# Autodesk Inventor assembly: assembly.rev5
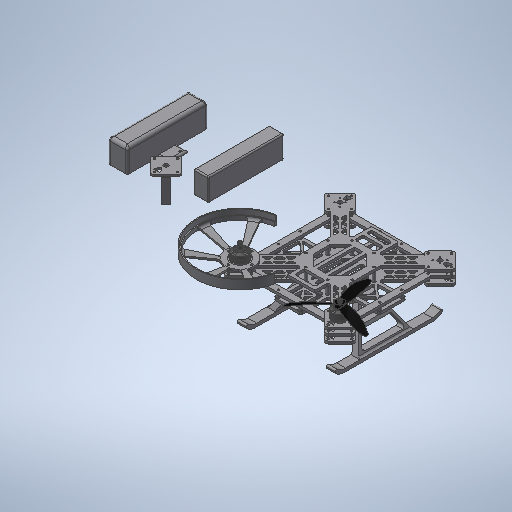
[picture p0: Inventor's stored thumbnail of the model, 512x512]
Saved by Autodesk Inventor 2025.2 (Build 292293000, 293)
## iProperties
Created: 2016-03-08
Part Number: assembly.rev5
Document SubType Name: Assembly
Designer: 200288284
Author: 200288284
## Documents named in this file (11)
- D:\UAV\机架\自制无人机\完整体.iam
- D:\UAV\机架\自制无人机\MOTOR_1806.iam
- D:\UAV\机架\自制无人机\Tri-Blade 5045 Propeller\Tri-Blade 5045 Propeller\5045 CCW.ipt
- D:\UAV\机架\自制无人机\电池.ipt
- D:\UAV\机架\自制无人机\Tri-Blade 5045 Propeller\Protection_for_2.5_inch_prop.ipt
- D:\UAV\机架\自制无人机\底板.ipt
- D:\UAV\机架\自制无人机\中版.ipt
- D:\UAV\机架\自制无人机\顶板.ipt
- D:\UAV\机架\自制无人机\起落架一体.ipt
- D:\UAV\机架\自制无人机\电池仓.ipt
- D:\UAV\机架\自制无人机\新起落架.ipt
## Components (13 placed, 10 different names)
1. 底板:1 — 配合:160, 配合:163, 配合:194, 配合:195, 表面齐平:1, 配合:196, 配合:197, 配合:199, 配合:200, 配合:201
2. 中版:1 — 配合:160, 配合:162, 配合:194, 配合:195
3. 顶板:1 — 配合:162, 配合:163, 配合:178, 配合:179, 配合:180, 配合:181, 配合:182, 配合:184, 配合:185, 配合:187, 配合:192, 配合:193
4. 电池:2 — 配合:192
5. MOTOR_1806:5 [sub-assembly] — 配合:180, 配合:181, 配合:183
6. Protection_for_2.5_inch_prop:5 — 配合:182, 配合:183, 配合:184
7. MOTOR_1806:8 [sub-assembly] — 配合:178, 配合:179, 配合:186, 配合:188, 配合:189
8. Protection_for_2.5_inch_prop:6 — 配合:185, 配合:186, 配合:187
9. 5045 CCW:5 — 配合:188, 配合:189
10. 电池仓:1 — 配合:193
11. 起落架一体:2
12. 新起落架:1 — 表面齐平:1, 配合:196, 配合:197
13. 新起落架:2 — 配合:199, 配合:200, 配合:201
## Relationships (25: Mate 24, Flush 1)
- 配合:160 [Mate]: 底板:1 ↔ 中版:1
- 配合:162 [Mate]: 中版:1 ↔ 顶板:1
- 配合:163 [Mate]: 底板:1 ↔ 顶板:1
- 配合:178 [Mate]: 顶板:1 ↔ MOTOR_1806:8
- 配合:179 [Mate]: 顶板:1 ↔ MOTOR_1806:8
- 配合:180 [Mate]: 顶板:1 ↔ MOTOR_1806:5
- 配合:181 [Mate]: 顶板:1 ↔ MOTOR_1806:5
- 配合:182 [Mate]: 顶板:1 ↔ Protection_for_2.5_inch_prop:5
- 配合:183 [Mate]: MOTOR_1806:5 ↔ Protection_for_2.5_inch_prop:5
- 配合:184 [Mate]: 顶板:1 ↔ Protection_for_2.5_inch_prop:5
- 配合:185 [Mate]: 顶板:1 ↔ Protection_for_2.5_inch_prop:6
- 配合:186 [Mate]: MOTOR_1806:8 ↔ Protection_for_2.5_inch_prop:6
- 配合:187 [Mate]: 顶板:1 ↔ Protection_for_2.5_inch_prop:6
- 配合:188 [Mate]: MOTOR_1806:8 ↔ 5045 CCW:5
- 配合:189 [Mate]: MOTOR_1806:8 ↔ 5045 CCW:5
- 配合:192 [Mate]: 顶板:1 ↔ 电池:2
- 配合:193 [Mate]: 顶板:1 ↔ 电池仓:1
- 配合:194 [Mate]: 底板:1 ↔ 中版:1
- 配合:195 [Mate]: 底板:1 ↔ 中版:1
- 表面齐平:1 [Flush]: 底板:1 ↔ 新起落架:1
- 配合:196 [Mate]: 底板:1 ↔ 新起落架:1
- 配合:197 [Mate]: 底板:1 ↔ 新起落架:1
- 配合:199 [Mate]: 底板:1 ↔ 新起落架:2
- 配合:200 [Mate]: 底板:1 ↔ 新起落架:2
- 配合:201 [Mate]: 底板:1 ↔ 新起落架:2
